# Autodesk Inventor assembly: SimulationWheelAssembly
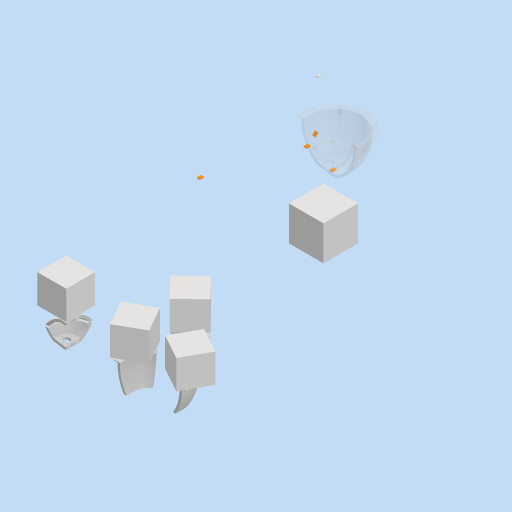
[picture p0: Inventor's stored thumbnail of the model, 512x512]
Saved by Autodesk Inventor 2023 (Build 270158000, 158)
## iProperties
Created: 2026-03-22
Part Number: SimulationWheelAssembly
Document SubType Name: Assembly
Designer: Nathann
Mass: 20175 g
Surface Area: 18221.2 cm^2
Volume: 20175 cm^3
Density: 1 g/cm^3
Author: Nathann
## Documents named in this file (16)
- C:\Users\Nathann\ClawdDrive\Objet3D\neodrive\neodrive-cad-ergonomic-v1\SimulationWheelAssembly.iam
- C:\Users\Nathann\ClawdDrive\Objet3D\neodrive\neodrive-cad-ergonomic-v1\prusaXL.ipt
- C:\Users\Nathann\ClawdDrive\Objet3D\neodrive\neodrive-cad-ergonomic-v1\ImprimanteDario.ipt
- C:\Users\Nathann\ClawdDrive\Objet3D\neodrive\neodrive-cad-ergonomic-v1\eggshellCorePrintedLeftA.ipt
- C:\Users\Nathann\ClawdDrive\Objet3D\neodrive\neodrive-cad-ergonomic-v1\eggshellCorePrintedLeftE.ipt
- C:\Users\Nathann\ClawdDrive\Objet3D\neodrive\neodrive-cad-ergonomic-v1\eggshellCorePrintedLeftF.ipt
- C:\Users\Nathann\ClawdDrive\Objet3D\neodrive\neodrive-cad-ergonomic-v1\eggshellCorePrintedLeftG.ipt
- C:\Users\Nathann\ClawdDrive\Objet3D\neodrive\neodrive-cad-ergonomic-v1\eggshellCorePrintedLeftH.ipt
- C:\Users\Nathann\ClawdDrive\Objet3D\neodrive\neodrive-cad-ergonomic-v1\peg.ipt
- C:\Users\Nathann\ClawdDrive\Objet3D\neodrive\neodrive-cad-ergonomic-v1\pegshort.ipt
- C:\Users\Nathann\ClawdDrive\Objet3D\neodrive\neodrive-cad-ergonomic-v1\SimulationWheelAssembly\AIP\FEA\fdktl59i8.fins
- C:\Users\Nathann\ClawdDrive\Objet3D\neodrive\neodrive-cad-ergonomic-v1\SimulationWheelAssembly\AIP\FEA\fdktl59i8.fsat
- C:\Users\Nathann\ClawdDrive\Objet3D\neodrive\neodrive-cad-ergonomic-v1\SimulationWheelAssembly\AIP\FEA\fdktl59j4.ftes
- C:\Users\Nathann\ClawdDrive\Objet3D\neodrive\neodrive-cad-ergonomic-v1\SimulationWheelAssembly\AIP\FEA\fdktl59j4.fwiz
- C:\Users\Nathann\ClawdDrive\Objet3D\neodrive\neodrive-cad-ergonomic-v1\SimulationWheelAssembly\AIP\FEA\fdktl59k0.fmsh
- C:\Users\Nathann\ClawdDrive\Objet3D\neodrive\neodrive-cad-ergonomic-v1\SimulationWheelAssembly\AIP\FEA\fdktl59k1.fres
## Components (20 placed, 9 different names)
1. prusaXL:1
2. ImprimanteDario:1
3. eggshellCorePrintedLeftA:1 — Mate:1, Mate:2, Mate:3, Mate:4, Mate:5, Mate:6, Mate:7, Flush:1, Mate:8, Flush:2, Mate:9, Tangent:1, Flush:3, Mate:11
4. eggshellCorePrintedLeftE:1 — Flush:1, Mate:8, Flush:2, Mate:10, Flush:4, Tangent:2, Tangent:3
5. eggshellCorePrintedLeftF:1 — Mate:10, Flush:4, Tangent:2, Mate:12
6. eggshellCorePrintedLeftG:1 — Mate:11, Tangent:3, Mate:12
7. eggshellCorePrintedLeftH:1 — Mate:9, Tangent:1, Flush:3
8. eggshellCorePrintedLeftA:2
9. eggshellCorePrintedLeftE:2
10. eggshellCorePrintedLeftF:2
11. eggshellCorePrintedLeftG:2
12. eggshellCorePrintedLeftH:2
13. prusaXL:2
14. prusaXL:3
15. prusaXL:4
16. peg:1
17. peg:2 — Mate:1, Mate:2, Mate:3
18. peg:3 — Mate:4, Mate:5
19. peg:4 — Mate:6, Mate:7
20. pegshort:1
## Relationships (19: Mate 12, Flush 4, Tangent 3)
- Mate:1: eggshellCorePrintedLeftA:1 ↔ peg:2
- Mate:2: eggshellCorePrintedLeftA:1 ↔ peg:2
- Mate:3: eggshellCorePrintedLeftA:1 ↔ peg:2
- Mate:4: eggshellCorePrintedLeftA:1 ↔ peg:3
- Mate:5: eggshellCorePrintedLeftA:1 ↔ peg:3
- Mate:6: eggshellCorePrintedLeftA:1 ↔ peg:4
- Mate:7: eggshellCorePrintedLeftA:1 ↔ peg:4
- Flush:1: eggshellCorePrintedLeftA:1 ↔ eggshellCorePrintedLeftE:1
- Mate:8: eggshellCorePrintedLeftA:1 ↔ eggshellCorePrintedLeftE:1
- Flush:2: eggshellCorePrintedLeftA:1 ↔ eggshellCorePrintedLeftE:1
- Mate:9: eggshellCorePrintedLeftA:1 ↔ eggshellCorePrintedLeftH:1
- Tangent:1: eggshellCorePrintedLeftA:1 ↔ eggshellCorePrintedLeftH:1
- Flush:3: eggshellCorePrintedLeftA:1 ↔ eggshellCorePrintedLeftH:1
- Mate:10: eggshellCorePrintedLeftE:1 ↔ eggshellCorePrintedLeftF:1
- Flush:4: eggshellCorePrintedLeftE:1 ↔ eggshellCorePrintedLeftF:1
- Tangent:2: eggshellCorePrintedLeftE:1 ↔ eggshellCorePrintedLeftF:1
- Mate:11: eggshellCorePrintedLeftA:1 ↔ eggshellCorePrintedLeftG:1
- Tangent:3: eggshellCorePrintedLeftE:1 ↔ eggshellCorePrintedLeftG:1
- Mate:12: eggshellCorePrintedLeftF:1 ↔ eggshellCorePrintedLeftG:1
## Named parameters: sa_0 = 300000, sa_1 = 0 mm, sa_2 = -700 mm, sa_3 = 0 mm, sa_4 = 300000
note: some values were not read from the file. Shown as the stored number, unit unknown: "sa_0", "sa_4".
